# Autodesk Inventor assembly: アームアセンブリ6
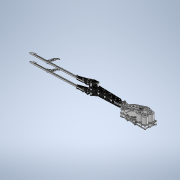
[picture p0: Inventor's stored thumbnail of the model, 180x180]
Saved by Autodesk Inventor 2020 (Build 240168000, 168)
## iProperties
Created: 2019-09-05
Part Number: アームアセンブリ6
Document SubType Name: Assembly
Designer: 雪村
Mass: 846.408 g
Surface Area: 2303.91 cm^2
Volume: 290.332 cm^3
Density: 2.91532 g/cm^3
Author: 雪村
## Documents named in this file (46)
- G:\マイドライブ\かわさき班共有ファイル\02.設計データ\2020年\雪村\2020年機体完成版\部品\アームアセンブリ6.iam
- G:\マイドライブ\かわさき班共有ファイル\02.設計データ\2020年\雪村\2020年機体完成版\部品\アームフレーム8.1.ipt
- G:\マイドライブ\かわさき班共有ファイル\02.設計データ\2020年\雪村\2020年機体完成版\部品\アームフレーム8.2.ipt
- G:\マイドライブ\かわさき班共有ファイル\02.設計データ\2020年\雪村\2020年機体完成版\パーツ\RS-380.iam
- G:\マイドライブ\かわさき班共有ファイル\02.設計データ\2020年\雪村\2020年機体完成版\パーツ\ベアリングフランジ付き0615.5t.ipt
- G:\マイドライブ\かわさき班共有ファイル\02.設計データ\2020年\雪村\2020年機体完成版\パーツ\ベアリングフランジ付き040904.ipt
- G:\マイドライブ\かわさき班共有ファイル\02.設計データ\2020年\雪村\2020年機体完成版\部品\多段ギアm1.z57,m2.z8.ipt
- G:\マイドライブ\かわさき班共有ファイル\02.設計データ\2020年\雪村\2020年機体完成版\部品\歯車m2.z41(z8).ipt
- G:\マイドライブ\かわさき班共有ファイル\02.設計データ\2020年\雪村\2020年機体完成版\部品\アーム中間節カム1.ipt
- G:\マイドライブ\かわさき班共有ファイル\02.設計データ\2020年\雪村\2020年機体完成版\パーツ\オイレスフランジ付き151703.ipt
- G:\マイドライブ\かわさき班共有ファイル\02.設計データ\2020年\雪村\2020年機体完成版\部品\アーム駆動節1.ipt
- G:\マイドライブ\かわさき班共有ファイル\02.設計データ\2020年\雪村\2020年機体完成版\部品\アーム中間節カム2.ipt
- G:\マイドライブ\かわさき班共有ファイル\02.設計データ\2020年\雪村\2020年機体完成版\部品\アーム揺動節2.ipt
- G:\マイドライブ\かわさき班共有ファイル\02.設計データ\2020年\雪村\2020年機体完成版\部品\アーム中間節2.1.ipt
- G:\マイドライブ\かわさき班共有ファイル\02.設計データ\2020年\雪村\2020年機体完成版\部品\アーム中間節2.2.ipt
- G:\マイドライブ\かわさき班共有ファイル\02.設計データ\2020年\雪村\2020年機体完成版\パーツ\オイレスフランジ付き081003.ipt
- G:\マイドライブ\かわさき班共有ファイル\02.設計データ\2020年\雪村\2020年機体完成版\パーツ\ワッシャー8.1,14,1t.ipt
- G:\マイドライブ\かわさき班共有ファイル\02.設計データ\2020年\雪村\2020年機体完成版\パーツ\オイレスフランジ付き081006.ipt
- G:\マイドライブ\かわさき班共有ファイル\02.設計データ\2020年\雪村\2020年機体完成版\部品\アーム軸抑え3.ipt
- G:\マイドライブ\かわさき班共有ファイル\02.設計データ\2020年\雪村\2020年機体完成版\パーツ\スペーサーm4,06.ipt
- G:\マイドライブ\かわさき班共有ファイル\02.設計データ\2020年\雪村\2020年機体完成版\パーツ\ナイロンナットm4.ipt
- G:\マイドライブ\かわさき班共有ファイル\02.設計データ\2020年\雪村\2020年機体完成版\パーツ\ネジ鍋m4,30.ipt
- G:\マイドライブ\かわさき班共有ファイル\02.設計データ\2020年\雪村\2020年機体完成版\パーツ\ネジ鍋m4,08.ipt
- G:\マイドライブ\かわさき班共有ファイル\02.設計データ\2020年\雪村\2020年機体完成版\パーツ\ネジ鍋m4,14.ipt
- G:\マイドライブ\かわさき班共有ファイル\02.設計データ\2020年\雪村\2020年機体完成版\パーツ\スペーサーm4,14.ipt
- G:\マイドライブ\かわさき班共有ファイル\02.設計データ\2020年\雪村\2020年機体完成版\パーツ\オイレス081004.ipt
- G:\マイドライブ\かわさき班共有ファイル\02.設計データ\2020年\雪村\2020年機体完成版\パーツ\シムリング0608,0.5t.ipt
- G:\マイドライブ\かわさき班共有ファイル\02.設計データ\2020年\雪村\2020年機体完成版\パーツ\オイレスフランジ付き06080512,1t ドライメット.ipt
- G:\マイドライブ\かわさき班共有ファイル\02.設計データ\2020年\雪村\2020年機体完成版\パーツ\オイレスフランジ付き06080312,1t ドライメット.ipt
- G:\マイドライブ\かわさき班共有ファイル\02.設計データ\2020年\雪村\2020年機体完成版\部品\焼結ギアm0.5.z80,m1.z10.ipt
- G:\マイドライブ\かわさき班共有ファイル\02.設計データ\2020年\雪村\2020年機体完成版\パーツ\シムリング0406,0.5t.ipt
- G:\マイドライブ\かわさき班共有ファイル\02.設計データ\2020年\雪村\2020年機体完成版\パーツ\シムリング0407.4t自作.ipt
- G:\マイドライブ\かわさき班共有ファイル\02.設計データ\2020年\雪村\2020年機体完成版\パーツ\平行ピンΦ6.25.ipt
- G:\マイドライブ\かわさき班共有ファイル\02.設計データ\2020年\雪村\2020年機体完成版\パーツ\平行ピンΦ4.22.ipt
- G:\マイドライブ\かわさき班共有ファイル\02.設計データ\2020年\雪村\2020年機体完成版\パーツ\平行ピンΦ6.20 片雌ネジ.ipt
- G:\マイドライブ\かわさき班共有ファイル\02.設計データ\2020年\雪村\2020年機体完成版\パーツ\スペーサーm4,30.ipt
- G:\マイドライブ\かわさき班共有ファイル\02.設計データ\2020年\雪村\2020年機体完成版\パーツ\ネジ皿m4,08.ipt
- G:\マイドライブ\かわさき班共有ファイル\02.設計データ\2020年\雪村\2020年機体完成版\部品\アームユニット底板締結パーツ3.ipt
- G:\マイドライブ\かわさき班共有ファイル\02.設計データ\2020年\雪村\2020年機体完成版\パーツ\スペーサーm3,13.ipt
- D:\SRDC\SRDC\Inventor_2017\2018年機体\alternative\アーム詰め物1.ipt
- G:\マイドライブ\かわさき班共有ファイル\02.設計データ\2020年\雪村\2020年機体完成版\パーツ\スペーサーm3,16.ipt
- G:\マイドライブ\かわさき班共有ファイル\02.設計データ\2020年\雪村\2020年機体完成版\パーツ\ネジ鍋m3,08.ipt
- G:\マイドライブ\かわさき班共有ファイル\02.設計データ\2020年\雪村\2020年機体完成版\パーツ\ネジ鍋m2.6,06.ipt
- G:\マイドライブ\かわさき班共有ファイル\02.設計データ\2020年\雪村\2020年機体完成版\パーツ\ワッシャー6.2,14.0.5t.ipt
- G:\マイドライブ\かわさき班共有ファイル\02.設計データ\2020年\雪村\2020年機体完成版\パーツ\オイレスフランジ付き06080312.ipt
- G:\マイドライブ\かわさき班共有ファイル\02.設計データ\2020年\雪村\2020年機体完成版\部品\アーム先端ツイン1.iam
## Components (94 placed, 45 different names)
1. アームフレーム8.1:1 — メイト:1, 挿入:1, 挿入:2, 挿入:3, 挿入:4, メイト:2, メイト:3, メイト:4, メイト:5, 挿入:26, 挿入:27, 挿入:32, メイト:12, 挿入:38, 挿入:55, メイト:17, メイト:19, 挿入:57, 挿入:58, 挿入:59, 挿入:60, 挿入:61, 挿入:62, 挿入:72, 挿入:73, 挿入:74, 挿入:75, 挿入:76, 挿入:77, 挿入:85, 挿入:86, 挿入:87, 挿入:88, 挿入:89, 挿入:90, 挿入:91, 挿入:92, 挿入:94, 挿入:95
2. アームフレーム8.2:1 — 挿入:28, 挿入:29, 挿入:39, 挿入:52, 挿入:53, 挿入:54, メイト:18, 挿入:78, 挿入:80, 挿入:81, 挿入:82, 挿入:83, 挿入:84, 挿入:96, 挿入:97
3. RS-380:1 [sub-assembly] — 挿入:4, メイト:5
4. RS-380:2 [sub-assembly] — 挿入:3, メイト:4
5. RS-380:3 [sub-assembly] — 挿入:1, メイト:2
6. RS-380:4 [sub-assembly] — 挿入:2, メイト:3
7. ベアリングフランジ付き0615.5t:1 — 挿入:29, 挿入:47, 挿入:49
8. ベアリングフランジ付き0615.5t:2 — 挿入:26, 挿入:41
9. ベアリングフランジ付き040904:1 — 挿入:28, メイト:16, 挿入:48
10. ベアリングフランジ付き040904:2 — 挿入:27, メイト:15, 挿入:44
11. 多段ギアm1.z57,m2.z8:1 — 挿入:40, 挿入:46
12. 歯車m2.z41(z8):1 — メイト:12, 挿入:101
13. アーム中間節カム1:1 — 挿入:34, メイト:21, 挿入:101
14. オイレスフランジ付き151703:1
15. アーム駆動節1:1
16. アーム中間節カム2:1
17. アーム揺動節2:1 — メイト:13
18. アーム中間節2.1:1 — 挿入:35, 挿入:36, メイト:13, 挿入:68, 挿入:69
19. アーム中間節2.2:1 — 挿入:70, メイト:23
20. オイレスフランジ付き081003:1
21. ワッシャー8.1,14,1t:1
22. ワッシャー8.1,14,1t:2 — 挿入:33
23. オイレスフランジ付き081006:1
24. ワッシャー8.1,14,1t:3
25. アーム軸抑え3:1 — 挿入:37, メイト:14, 挿入:51
26. オイレスフランジ付き081003:2 — メイト:14
27. スペーサーm4,06:1
28. ナイロンナットm4:1
29. ナイロンナットm4:2
30. ネジ鍋m4,30:1
31. ネジ鍋m4,30:2 — メイト:21
32. ネジ鍋m4,08:1
33. ネジ鍋m4,14:1
34. ネジ鍋m4,14:2
35. オイレスフランジ付き081003:3 — 挿入:97
36. オイレスフランジ付き081003:4 — 挿入:95
37. スペーサーm4,14:1 — 挿入:32, 挿入:33, 挿入:37
38. オイレスフランジ付き151703:2 — 挿入:34, 挿入:35
39. オイレス081004:1 — 挿入:36
40. シムリング0608,0.5t:1 — 挿入:40, 挿入:41
41. オイレスフランジ付き06080512,1t ドライメット:1 — 挿入:39, 挿入:99
42. オイレスフランジ付き06080312,1t ドライメット:1 — 挿入:38, 挿入:50, 挿入:98
43. 焼結ギアm0.5.z80,m1.z10:1 — メイト:15, 挿入:42, 挿入:45, メイト:16
44. シムリング0406,0.5t:1 — 挿入:42
45. シムリング0407.4t自作:1 — 挿入:45
46. シムリング0406,0.5t:2 — 挿入:44
47. シムリング0608,0.5t:2 — 挿入:46, 挿入:47
48. 平行ピンΦ6.25:1 — 挿入:49
49. 平行ピンΦ4.22:1 — 挿入:48
50. 平行ピンΦ6.20 片雌ネジ:1 — 挿入:50
51. スペーサーm4,30:1 — 挿入:52
52. スペーサーm4,30:2 — 挿入:51
53. ネジ皿m4,08:1 — 挿入:55
54. ネジ鍋m4,14:3 — 挿入:53
55. ネジ鍋m4,14:4 — 挿入:54
56. アームユニット底板締結パーツ3:1 — メイト:17, メイト:18, メイト:19
57. スペーサーm3,13:1 — 挿入:57
58. スペーサーm3,13:2 — 挿入:58
59. スペーサーm3,13:3 — 挿入:60
60. スペーサーm3,13:4 — 挿入:61
61. スペーサーm3,13:5 — 挿入:62
62. スペーサーm3,13:6
63. スペーサーm3,13:7 — 挿入:59
64. アーム詰め物1:1 — 挿入:70
65. アーム詰め物1:2 — 挿入:68, 挿入:69
66. スペーサーm3,16:1
67. スペーサーm3,16:2 — 挿入:102
68. スペーサーm3,16:3 — メイト:23, メイト:24
69. ネジ鍋m3,08:1 — 挿入:78
70. ネジ鍋m3,08:2 — 挿入:96
71. ネジ鍋m3,08:3 — 挿入:80
72. ネジ鍋m3,08:4 — 挿入:81
73. ネジ鍋m3,08:5 — 挿入:82
74. ネジ鍋m3,08:6 — 挿入:83
75. ネジ鍋m3,08:7 — 挿入:84
76. ネジ鍋m3,08:8 — 挿入:76
77. ネジ鍋m3,08:9 — 挿入:75
78. ネジ鍋m3,08:10 — 挿入:73
79. ネジ鍋m3,08:11 — 挿入:72
80. ネジ鍋m3,08:12 — 挿入:74
81. ネジ鍋m3,08:13 — 挿入:94
82. ネジ鍋m3,08:14 — 挿入:77
83. ネジ鍋m2.6,06:1 — 挿入:89
84. ネジ鍋m2.6,06:2 — 挿入:86
85. ネジ鍋m2.6,06:3 — 挿入:88
86. ネジ鍋m2.6,06:4 — 挿入:85
87. ネジ鍋m2.6,06:5 — 挿入:92
88. ネジ鍋m2.6,06:6 — 挿入:91
89. ネジ鍋m2.6,06:7 — 挿入:87
90. ネジ鍋m2.6,06:8 — 挿入:90
91. ワッシャー6.2,14.0.5t:1 — 挿入:98
92. ワッシャー6.2,14.0.5t:2 — 挿入:100
93. オイレスフランジ付き06080312:1 — 挿入:99, 挿入:100
94. アーム先端ツイン1:1 [sub-assembly] — 挿入:102, メイト:24
## Relationships (113: Insert 92, Mate 21)
- メイト:1 [Mate] (48 mm): アームフレーム8.1:1
- 挿入:1 [Insert]: アームフレーム8.1:1 ↔ RS-380:3
- 挿入:2 [Insert]: アームフレーム8.1:1 ↔ RS-380:4
- 挿入:3 [Insert]: アームフレーム8.1:1 ↔ RS-380:2
- 挿入:4 [Insert]: アームフレーム8.1:1 ↔ RS-380:1
- メイト:2 [Mate]: アームフレーム8.1:1 ↔ RS-380:3
- メイト:3 [Mate]: アームフレーム8.1:1 ↔ RS-380:4
- メイト:4 [Mate]: アームフレーム8.1:1 ↔ RS-380:2
- メイト:5 [Mate]: アームフレーム8.1:1 ↔ RS-380:1
- [Insert]: アーム中間節カム1:1 ↔ アーム中間節カム2:1
- [Mate]: アーム中間節カム1:1 ↔ アーム中間節カム2:1
- [Insert]: アーム駆動節1:1 ↔ アーム中間節カム2:1
- [Insert]: アーム駆動節1:1 ↔ アーム中間節カム2:1
- [Insert]: オイレスフランジ付き151703:1 ↔ アーム中間節カム2:1
- [Insert]: アーム中間節2.1:1 ↔ アーム中間節2.2:1
- [Mate]: アーム中間節カム1:1 ↔ アーム中間節2.2:1
- [Insert]: オイレスフランジ付き081003:1 ↔ ワッシャー8.1,14,1t:1
- [Insert]: ワッシャー8.1,14,1t:1 ↔ ワッシャー8.1,14,1t:2
- [Insert]: オイレスフランジ付き081006:1 ↔ ワッシャー8.1,14,1t:3
- [Insert]: アーム揺動節2:1 ↔ オイレスフランジ付き081003:1
- [Insert]: アーム揺動節2:1 ↔ ワッシャー8.1,14,1t:3
- [Insert]: アーム駆動節1:1 ↔ オイレスフランジ付き081003:2
- [Insert]: アーム駆動節1:1 ↔ スペーサーm4,06:1
- [Mate]: アーム揺動節2:1 ↔ アーム中間節2.1:1
- [Insert]: アーム駆動節1:1 ↔ ナイロンナットm4:2
- [Insert]: アーム駆動節1:1 ↔ ナイロンナットm4:1
- [Mate]: アーム駆動節1:1 ↔ ナイロンナットm4:2
- [Mate]: アーム駆動節1:1 ↔ ナイロンナットm4:1
- [Insert]: 歯車m2.z41(z8):1 ↔ ネジ鍋m4,30:1
- [Insert]: 歯車m2.z41(z8):1 ↔ ネジ鍋m4,30:2
- [Insert]: アーム軸抑え3:1 ↔ ネジ鍋m4,08:1
- [Insert]: アーム軸抑え3:1 ↔ ネジ鍋m4,14:1
- [Insert]: アーム軸抑え3:1 ↔ ネジ鍋m4,14:2
- 挿入:26 [Insert]: アームフレーム8.1:1 ↔ ベアリングフランジ付き0615.5t:2
- 挿入:27 [Insert]: アームフレーム8.1:1 ↔ ベアリングフランジ付き040904:2
- 挿入:28 [Insert]: アームフレーム8.2:1 ↔ ベアリングフランジ付き040904:1
- 挿入:29 [Insert]: アームフレーム8.2:1 ↔ ベアリングフランジ付き0615.5t:1
- 挿入:32 [Insert]: アームフレーム8.1:1 ↔ スペーサーm4,14:1
- 挿入:33 [Insert]: ワッシャー8.1,14,1t:2 ↔ スペーサーm4,14:1
- メイト:12 [Mate]: アームフレーム8.1:1 ↔ 歯車m2.z41(z8):1
- 挿入:34 [Insert]: アーム中間節カム1:1 ↔ オイレスフランジ付き151703:2
- 挿入:35 [Insert]: アーム中間節2.1:1 ↔ オイレスフランジ付き151703:2
- 挿入:36 [Insert]: アーム中間節2.1:1 ↔ オイレス081004:1
- メイト:13 [Mate] (0.5 mm): アーム揺動節2:1 ↔ アーム中間節2.1:1
- 挿入:37 [Insert]: アーム軸抑え3:1 ↔ スペーサーm4,14:1
- メイト:14 [Mate]: アーム軸抑え3:1 ↔ オイレスフランジ付き081003:2
- 挿入:38 [Insert]: アームフレーム8.1:1 ↔ オイレスフランジ付き06080312,1t ドライメット:1
- 挿入:39 [Insert]: アームフレーム8.2:1 ↔ オイレスフランジ付き06080512,1t ドライメット:1
- 挿入:40 [Insert]: 多段ギアm1.z57,m2.z8:1 ↔ シムリング0608,0.5t:1
- 挿入:41 [Insert]: ベアリングフランジ付き0615.5t:2 ↔ シムリング0608,0.5t:1
- メイト:15 [Mate]: ベアリングフランジ付き040904:2 ↔ 焼結ギアm0.5.z80,m1.z10:1
- 挿入:42 [Insert]: 焼結ギアm0.5.z80,m1.z10:1 ↔ シムリング0406,0.5t:1
- [Insert]: シムリング0407.4t自作:1 ↔ シムリング0406,0.5t:2
- 挿入:44 [Insert]: ベアリングフランジ付き040904:2 ↔ シムリング0406,0.5t:2
- 挿入:45 [Insert]: 焼結ギアm0.5.z80,m1.z10:1 ↔ シムリング0407.4t自作:1
- 挿入:46 [Insert]: 多段ギアm1.z57,m2.z8:1 ↔ シムリング0608,0.5t:2
- 挿入:47 [Insert]: ベアリングフランジ付き0615.5t:1 ↔ シムリング0608,0.5t:2
- メイト:16 [Mate]: ベアリングフランジ付き040904:1 ↔ 焼結ギアm0.5.z80,m1.z10:1
- 挿入:48 [Insert] (-0.5 mm): ベアリングフランジ付き040904:1 ↔ 平行ピンΦ4.22:1
- 挿入:49 [Insert] (-1 mm): ベアリングフランジ付き0615.5t:1 ↔ 平行ピンΦ6.25:1
- 挿入:50 [Insert]: オイレスフランジ付き06080312,1t ドライメット:1 ↔ 平行ピンΦ6.20 片雌ネジ:1
- 挿入:51 [Insert]: アーム軸抑え3:1 ↔ スペーサーm4,30:2
- 挿入:52 [Insert]: アームフレーム8.2:1 ↔ スペーサーm4,30:1
- 挿入:53 [Insert]: アームフレーム8.2:1 ↔ ネジ鍋m4,14:3
- 挿入:54 [Insert]: アームフレーム8.2:1 ↔ ネジ鍋m4,14:4
- 挿入:55 [Insert]: アームフレーム8.1:1 ↔ ネジ皿m4,08:1
- メイト:17 [Mate]: アームフレーム8.1:1 ↔ アームユニット底板締結パーツ3:1
- メイト:18 [Mate]: アームフレーム8.2:1 ↔ アームユニット底板締結パーツ3:1
- メイト:19 [Mate]: アームフレーム8.1:1 ↔ アームユニット底板締結パーツ3:1
- 挿入:57 [Insert]: アームフレーム8.1:1 ↔ スペーサーm3,13:1
- 挿入:58 [Insert]: アームフレーム8.1:1 ↔ スペーサーm3,13:2
- 挿入:59 [Insert]: アームフレーム8.1:1 ↔ スペーサーm3,13:7
- 挿入:60 [Insert]: アームフレーム8.1:1 ↔ スペーサーm3,13:3
- 挿入:61 [Insert]: アームフレーム8.1:1 ↔ スペーサーm3,13:4
- 挿入:62 [Insert]: アームフレーム8.1:1 ↔ スペーサーm3,13:5
- [Insert] (-1 mm): アーム詰め物1:1 ↔ スペーサーm3,16:3
- [Insert] (-1 mm): アーム詰め物1:1 ↔ スペーサーm3,16:1
- [Insert] (-1 mm): アーム詰め物1:1 ↔ スペーサーm3,16:2
- 挿入:68 [Insert]: アーム中間節2.1:1 ↔ アーム詰め物1:2
- 挿入:69 [Insert]: アーム中間節2.1:1 ↔ アーム詰め物1:2
- 挿入:70 [Insert]: アーム中間節2.2:1 ↔ アーム詰め物1:1
- 挿入:72 [Insert]: アームフレーム8.1:1 ↔ ネジ鍋m3,08:11
- 挿入:73 [Insert]: アームフレーム8.1:1 ↔ ネジ鍋m3,08:10
- 挿入:74 [Insert]: アームフレーム8.1:1 ↔ ネジ鍋m3,08:12
- 挿入:75 [Insert]: アームフレーム8.1:1 ↔ ネジ鍋m3,08:9
- 挿入:76 [Insert]: アームフレーム8.1:1 ↔ ネジ鍋m3,08:8
- 挿入:77 [Insert]: アームフレーム8.1:1 ↔ ネジ鍋m3,08:14
- 挿入:78 [Insert]: アームフレーム8.2:1 ↔ ネジ鍋m3,08:1
- 挿入:80 [Insert]: アームフレーム8.2:1 ↔ ネジ鍋m3,08:3
- 挿入:81 [Insert]: アームフレーム8.2:1 ↔ ネジ鍋m3,08:4
- 挿入:82 [Insert]: アームフレーム8.2:1 ↔ ネジ鍋m3,08:5
- 挿入:83 [Insert]: アームフレーム8.2:1 ↔ ネジ鍋m3,08:6
- 挿入:84 [Insert]: アームフレーム8.2:1 ↔ ネジ鍋m3,08:7
- 挿入:85 [Insert]: アームフレーム8.1:1 ↔ ネジ鍋m2.6,06:4
- 挿入:86 [Insert]: アームフレーム8.1:1 ↔ ネジ鍋m2.6,06:2
- 挿入:87 [Insert]: アームフレーム8.1:1 ↔ ネジ鍋m2.6,06:7
- 挿入:88 [Insert]: アームフレーム8.1:1 ↔ ネジ鍋m2.6,06:3
- 挿入:89 [Insert]: アームフレーム8.1:1 ↔ ネジ鍋m2.6,06:1
- 挿入:90 [Insert]: アームフレーム8.1:1 ↔ ネジ鍋m2.6,06:8
- 挿入:91 [Insert]: アームフレーム8.1:1 ↔ ネジ鍋m2.6,06:6
- 挿入:92 [Insert]: アームフレーム8.1:1 ↔ ネジ鍋m2.6,06:5
- 挿入:94 [Insert]: アームフレーム8.1:1 ↔ ネジ鍋m3,08:13
- 挿入:95 [Insert]: アームフレーム8.1:1 ↔ オイレスフランジ付き081003:4
- 挿入:96 [Insert]: アームフレーム8.2:1 ↔ ネジ鍋m3,08:2
- 挿入:97 [Insert]: アームフレーム8.2:1 ↔ オイレスフランジ付き081003:3
- 挿入:98 [Insert]: オイレスフランジ付き06080312,1t ドライメット:1 ↔ ワッシャー6.2,14.0.5t:1
- 挿入:99 [Insert]: オイレスフランジ付き06080512,1t ドライメット:1 ↔ オイレスフランジ付き06080312:1
- 挿入:100 [Insert]: ワッシャー6.2,14.0.5t:2 ↔ オイレスフランジ付き06080312:1
- メイト:21 [Mate]: アーム中間節カム1:1 ↔ ネジ鍋m4,30:2
- 挿入:101 [Insert]: 歯車m2.z41(z8):1 ↔ アーム中間節カム1:1
- メイト:23 [Mate]: アーム中間節2.2:1 ↔ スペーサーm3,16:3
- 挿入:102 [Insert]: スペーサーm3,16:2 ↔ アーム先端ツイン1:1
- メイト:24 [Mate]: スペーサーm3,16:3 ↔ アーム先端ツイン1:1
## Named parameters: d64_d62 = 0 mm, d96_d91 = -1 mm, d104_d92 = -1 mm, d105_d93 = -1 mm
